# Autodesk Inventor assembly: mearm 期末組合
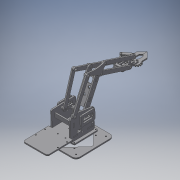
[picture p0: Inventor's stored thumbnail of the model, 180x180]
Saved by Autodesk Inventor 2019 (Build 230136000, 136)
## iProperties
Created: 2022-01-10
Part Number: mearm 期末組合
Material: 一般
Document SubType Name: Assembly
Designer: 10617
Author: 10617
## Documents named in this file (31)
- E:\cad2021\data\tmp\cad2021_hw\downloads\meARM\meARM_Inventor\HW1_mearm零組件\HW1_mearm組合.iam
- E:\cad2021\data\tmp\cad2021_hw\downloads\meARM\meARM_Inventor\HW1_mearm零組件\1.ipt
- E:\cad2021\data\tmp\cad2021_hw\downloads\meARM\meARM_Inventor\HW1_mearm零組件\2.ipt
- E:\cad2021\data\tmp\cad2021_hw\downloads\meARM\meARM_Inventor\HW1_mearm零組件\3.ipt
- E:\cad2021\data\tmp\cad2021_hw\downloads\meARM\meARM_Inventor\HW1_mearm零組件\4.ipt
- E:\cad2021\data\tmp\cad2021_hw\downloads\meARM\meARM_Inventor\HW1_mearm零組件\5.ipt
- E:\cad2021\data\tmp\cad2021_hw\downloads\meARM\meARM_Inventor\HW1_mearm零組件\6.ipt
- E:\cad2021\data\tmp\cad2021_hw\downloads\meARM\meARM_Inventor\HW1_mearm零組件\7.ipt
- E:\cad2021\data\tmp\cad2021_hw\downloads\meARM\meARM_Inventor\HW1_mearm零組件\8.ipt
- E:\cad2021\data\tmp\cad2021_hw\downloads\meARM\meARM_Inventor\HW1_mearm零組件\9.ipt
- E:\cad2021\data\tmp\cad2021_hw\downloads\meARM\meARM_Inventor\HW1_mearm零組件\10.ipt
- E:\cad2021\data\tmp\cad2021_hw\downloads\meARM\meARM_Inventor\HW1_mearm零組件\11.ipt
- E:\cad2021\data\tmp\cad2021_hw\downloads\meARM\meARM_Inventor\HW1_mearm零組件\12.ipt
- E:\cad2021\data\tmp\cad2021_hw\downloads\meARM\meARM_Inventor\HW1_mearm零組件\13.ipt
- E:\cad2021\data\tmp\cad2021_hw\downloads\meARM\meARM_Inventor\HW1_mearm零組件\14.ipt
- E:\cad2021\data\tmp\cad2021_hw\downloads\meARM\meARM_Inventor\HW1_mearm零組件\15.ipt
- E:\cad2021\data\tmp\cad2021_hw\downloads\meARM\meARM_Inventor\HW1_mearm零組件\16.ipt
- E:\cad2021\data\tmp\cad2021_hw\downloads\meARM\meARM_Inventor\HW1_mearm零組件\17.ipt
- E:\cad2021\data\tmp\cad2021_hw\downloads\meARM\meARM_Inventor\HW1_mearm零組件\18.ipt
- E:\cad2021\data\tmp\cad2021_hw\downloads\meARM\meARM_Inventor\HW1_mearm零組件\19.ipt
- E:\cad2021\data\tmp\cad2021_hw\downloads\meARM\meARM_Inventor\HW1_mearm零組件\20.ipt
- E:\cad2021\data\tmp\cad2021_hw\downloads\meARM\meARM_Inventor\HW1_mearm零組件\21.ipt
- E:\cad2021\data\tmp\cad2021_hw\downloads\meARM\meARM_Inventor\HW1_mearm零組件\22.ipt
- E:\cad2021\data\tmp\cad2021_hw\downloads\meARM\meARM_Inventor\HW1_mearm零組件\24.ipt
- E:\cad2021\data\tmp\cad2021_hw\downloads\meARM\meARM_Inventor\HW1_mearm零組件\25.ipt
- E:\cad2021\data\tmp\cad2021_hw\downloads\meARM\meARM_Inventor\HW1_mearm零組件\26.ipt
- E:\cad2021\data\tmp\cad2021_hw\downloads\meARM\meARM_Inventor\HW1_mearm零組件\27.ipt
- E:\cad2021\data\tmp\cad2021_hw\downloads\meARM\meARM_Inventor\HW1_mearm零組件\齒輪.ipt
- E:\cad2021\data\tmp\cad2021_hw\downloads\meARM\meARM_Inventor\HW1_mearm零組件\齒輪2.ipt
- E:\cad2021\data\tmp\cad2021_hw\downloads\meARM\meARM_Inventor\HW1_mearm零組件\23.ipt
- E:\cad2021\data\tmp\cad2021_hw\downloads\meARM\meARM_Inventor\HW1_mearm零組件\軸.ipt
## Components (48 placed, 30 different names)
1. 1:1 — 貼合:105, 貼合:108, 貼合:110, 貼合:117, 齊平:26, 貼合:166, 齊平:33
2. 2:1 — 貼合:106, 貼合:107, 貼合:109, 貼合:111, 貼合:112, 貼合:113, 齊平:22
3. 3:1 — 貼合:101, 貼合:102, 貼合:103, 貼合:104
4. 4:1 — 貼合:119, 貼合:120, 貼合:141
5. 5:1 — 貼合:99, 貼合:100, 貼合:114, 貼合:115, 貼合:163, 齊平:30, 齊平:31
6. 6:1 — 齊平:1, 貼合:1, 貼合:2, 貼合:3, 角度:2, 齊平:3, 貼合:77
7. 7:1 — 角度:2, 齊平:3, 齊平:4, 齊平:5
8. 8:1 — 貼合:86, 貼合:87, 貼合:88
9. 9:1 — 貼合:92, 貼合:93, 貼合:94, 貼合:95, 齊平:14, 貼合:96, 齊平:15
10. 10:1 — 貼合:84, 貼合:85, 齊平:13
11. 11:1 — 貼合:77, 齊平:12, 貼合:78, 貼合:79, 貼合:80, 貼合:81, 貼合:82, 貼合:83, 貼合:165, 齊平:32
12. 12:1 — 貼合:105, 貼合:106, 貼合:107, 貼合:108, 貼合:109, 貼合:110
13. 13:1 — 貼合:103, 貼合:104, 貼合:116, 貼合:118, 貼合:119, 貼合:120, 貼合:156, 齊平:23, 貼合:158, 齊平:25, 貼合:160, 齊平:27
14. 14:1 — 貼合:81, 貼合:82, 貼合:83, 貼合:85, 齊平:13, 貼合:86, 貼合:87, 貼合:88, 貼合:92, 貼合:93, 貼合:94
15. 15:1 — 貼合:116, 貼合:117, 貼合:118, 貼合:140, 貼合:157, 齊平:24
16. 16:1 — 貼合:78, 貼合:79, 貼合:80, 貼合:84, 貼合:89, 貼合:90, 貼合:91, 貼合:101, 貼合:102, 貼合:161, 齊平:28
17. 17:1 — 貼合:89, 貼合:90, 貼合:91
18. 18:1 — 貼合:123, 貼合:125, 貼合:127, 貼合:129, 貼合:142, 貼合:143
19. 19:1 — 貼合:136, 貼合:137, 貼合:139, 貼合:143, 貼合:148, 齊平:17
20. 20:1 — 貼合:97, 貼合:98, 貼合:99, 貼合:100, 貼合:162, 齊平:29, 貼合:164
21. 21:1 — 貼合:95, 齊平:14, 貼合:96, 貼合:97, 貼合:98, 貼合:111, 貼合:112
22. 22:1 — 齊平:1, 貼合:1, 貼合:2, 貼合:3, 齊平:4, 齊平:5, 齊平:12, 齊平:15
23. 24:1 — 貼合:127, 貼合:128, 貼合:129, 貼合:141, 貼合:142, 貼合:154, 齊平:21
24. 25:1 — 貼合:134, 貼合:135, 貼合:136, 貼合:137, 貼合:149, 貼合:150, 貼合:151, 齊平:18
25. 26:1 — 貼合:122, 貼合:123, 貼合:124, 貼合:125, 貼合:126, 貼合:139, 貼合:145, 貼合:146
26. 27:1 — 貼合:113, 貼合:114, 貼合:115, 貼合:140, 貼合:145, 貼合:146, 貼合:147, 齊平:16, 貼合:155
27. 齒輪:1 — 貼合:132, 貼合:133, 貼合:134, 貼合:135, 相切:1
28. 齒輪2:1 — 貼合:130, 貼合:131, 相切:1
29. 23:1 — 貼合:122, 貼合:124, 貼合:126, 貼合:128, 貼合:130, 貼合:131, 貼合:132, 貼合:133, 貼合:152, 齊平:19, 貼合:153, 齊平:20
30. 軸:1 — 貼合:148, 齊平:17
31. 軸:2 — 貼合:149, 貼合:150
32. 軸:3 — 貼合:151, 齊平:18
33. 軸:4 — 貼合:154, 齊平:21
34. 軸:5 — 貼合:157, 齊平:24
35. 軸:6 — 貼合:158, 齊平:25, 貼合:159
36. 軸:7 — 貼合:160, 齊平:27
37. 軸:8 — 貼合:164, 齊平:31
38. 軸:9 — 貼合:153, 齊平:20
39. 軸:10 — 貼合:161, 齊平:28
40. 軸:11 — 貼合:152, 齊平:19
41. 軸:12 — 貼合:163, 齊平:30
42. 軸:13 — 貼合:165, 齊平:32
43. 軸:14 — 貼合:166, 齊平:33
44. 軸:15 — 貼合:162, 齊平:29
45. 軸:16 — 貼合:159, 齊平:26
46. 軸:17 — 貼合:156, 齊平:23
47. 軸:18 — 貼合:155, 齊平:22
48. 軸:19 — 貼合:147, 齊平:16
## Relationships (118: Mate 90, Flush 26, Angle 1, Tangent 1)
- 齊平:1 [Flush] (13 mm): 6:1 ↔ 22:1
- 貼合:1 [Mate]: 6:1 ↔ 22:1
- 貼合:2 [Mate]: 6:1 ↔ 22:1
- 貼合:3 [Mate]: 6:1 ↔ 22:1
- 角度:2 [Angle] (0 deg): 6:1 ↔ 7:1
- 齊平:3 [Flush] (-7.63 mm): 6:1 ↔ 7:1
- 齊平:4 [Flush]: 7:1 ↔ 22:1
- 齊平:5 [Flush]: 7:1 ↔ 22:1
- 貼合:77 [Mate] (-27.48 mm): 6:1 ↔ 11:1
- 齊平:12 [Flush]: 11:1 ↔ 22:1
- 貼合:78 [Mate]: 11:1 ↔ 16:1
- 貼合:79 [Mate]: 11:1 ↔ 16:1
- 貼合:80 [Mate]: 11:1 ↔ 16:1
- 貼合:81 [Mate]: 11:1 ↔ 14:1
- 貼合:82 [Mate]: 11:1 ↔ 14:1
- 貼合:83 [Mate]: 11:1 ↔ 14:1
- 貼合:84 [Mate]: 10:1 ↔ 16:1
- 貼合:85 [Mate]: 10:1 ↔ 14:1
- 齊平:13 [Flush]: 10:1 ↔ 14:1
- 貼合:86 [Mate]: 8:1 ↔ 14:1
- 貼合:87 [Mate]: 8:1 ↔ 14:1
- 貼合:88 [Mate] (2.37 mm): 8:1 ↔ 14:1
- 貼合:89 [Mate]: 16:1 ↔ 17:1
- 貼合:90 [Mate]: 16:1 ↔ 17:1
- 貼合:91 [Mate] (2.37 mm): 16:1 ↔ 17:1
- 貼合:92 [Mate]: 9:1 ↔ 14:1
- 貼合:93 [Mate]: 9:1 ↔ 14:1
- 貼合:94 [Mate]: 9:1 ↔ 14:1
- 貼合:95 [Mate]: 9:1 ↔ 21:1
- 齊平:14 [Flush]: 9:1 ↔ 21:1
- 貼合:96 [Mate]: 9:1 ↔ 21:1
- 貼合:97 [Mate]: 20:1 ↔ 21:1
- 貼合:98 [Mate] (5 mm): 20:1 ↔ 21:1
- 貼合:99 [Mate]: 5:1 ↔ 20:1
- 貼合:100 [Mate] (1.5 mm): 5:1 ↔ 20:1
- 貼合:101 [Mate]: 3:1 ↔ 16:1
- 貼合:102 [Mate]: 3:1 ↔ 16:1
- 貼合:103 [Mate]: 3:1 ↔ 13:1
- 貼合:104 [Mate]: 3:1 ↔ 13:1
- 貼合:105 [Mate]: 1:1 ↔ 12:1
- 貼合:106 [Mate]: 2:1 ↔ 12:1
- 貼合:107 [Mate]: 2:1 ↔ 12:1
- 貼合:108 [Mate]: 1:1 ↔ 12:1
- 貼合:109 [Mate]: 2:1 ↔ 12:1
- 貼合:110 [Mate]: 1:1 ↔ 12:1
- 貼合:111 [Mate]: 2:1 ↔ 21:1
- 貼合:112 [Mate] (0.5 mm): 2:1 ↔ 21:1
- 貼合:113 [Mate]: 2:1 ↔ 27:1
- 貼合:114 [Mate]: 5:1 ↔ 27:1
- 貼合:115 [Mate]: 5:1 ↔ 27:1
- 貼合:116 [Mate]: 13:1 ↔ 15:1
- 貼合:117 [Mate]: 1:1 ↔ 15:1
- 貼合:118 [Mate]: 13:1 ↔ 15:1
- 貼合:119 [Mate]: 4:1 ↔ 13:1
- 貼合:120 [Mate]: 4:1 ↔ 13:1
- 貼合:122 [Mate]: 26:1 ↔ 23:1
- 貼合:123 [Mate]: 18:1 ↔ 26:1
- 貼合:124 [Mate]: 26:1 ↔ 23:1
- 貼合:125 [Mate]: 18:1 ↔ 26:1
- 貼合:126 [Mate]: 26:1 ↔ 23:1
- 貼合:127 [Mate]: 18:1 ↔ 24:1
- 貼合:128 [Mate]: 24:1 ↔ 23:1
- 貼合:129 [Mate]: 18:1 ↔ 24:1
- 齊平:15 [Flush] (6.88 mm): 9:1 ↔ 22:1
- 貼合:130 [Mate]: 齒輪2:1 ↔ 23:1
- 貼合:131 [Mate]: 齒輪2:1 ↔ 23:1
- 貼合:132 [Mate]: 齒輪:1 ↔ 23:1
- 貼合:133 [Mate]: 齒輪:1 ↔ 23:1
- 貼合:134 [Mate]: 25:1 ↔ 齒輪:1
- 貼合:135 [Mate]: 25:1 ↔ 齒輪:1
- 貼合:136 [Mate]: 19:1 ↔ 25:1
- 貼合:137 [Mate] (4.48 mm): 19:1 ↔ 25:1
- 貼合:139 [Mate] (-12 mm): 19:1 ↔ 26:1
- 貼合:140 [Mate]: 15:1 ↔ 27:1
- 貼合:141 [Mate]: 4:1 ↔ 24:1
- 貼合:142 [Mate]: 18:1 ↔ 24:1
- 貼合:143 [Mate] (-11 mm): 18:1 ↔ 19:1
- 貼合:145 [Mate]: 26:1 ↔ 27:1
- 貼合:146 [Mate] (1 mm): 26:1 ↔ 27:1
- 貼合:147 [Mate]: 27:1 ↔ 軸:19
- 齊平:16 [Flush] (-4 mm): 27:1 ↔ 軸:19
- 相切:1 [Tangent]: 齒輪:1 ↔ 齒輪2:1
- 貼合:148 [Mate]: 19:1 ↔ 軸:1
- 齊平:17 [Flush] (-2 mm): 19:1 ↔ 軸:1
- 貼合:149 [Mate]: 25:1 ↔ 軸:2
- 貼合:150 [Mate] (1 mm): 25:1 ↔ 軸:2
- 貼合:151 [Mate]: 25:1 ↔ 軸:3
- 齊平:18 [Flush] (-2 mm): 25:1 ↔ 軸:3
- 貼合:152 [Mate]: 23:1 ↔ 軸:11
- 齊平:19 [Flush] (-2 mm): 23:1 ↔ 軸:11
- 貼合:153 [Mate]: 23:1 ↔ 軸:9
- 齊平:20 [Flush] (-2 mm): 23:1 ↔ 軸:9
- 貼合:154 [Mate]: 24:1 ↔ 軸:4
- 齊平:21 [Flush] (-3 mm): 24:1 ↔ 軸:4
- 貼合:155 [Mate]: 27:1 ↔ 軸:18
- 齊平:22 [Flush] (-1 mm): 2:1 ↔ 軸:18
- 貼合:156 [Mate]: 13:1 ↔ 軸:17
- 齊平:23 [Flush] (2 mm): 13:1 ↔ 軸:17
- 貼合:157 [Mate]: 15:1 ↔ 軸:5
- 齊平:24 [Flush] (-2 mm): 15:1 ↔ 軸:5
- 貼合:158 [Mate]: 13:1 ↔ 軸:6
- 齊平:25 [Flush] (-2 mm): 13:1 ↔ 軸:6
- 貼合:159 [Mate]: 軸:6 ↔ 軸:16
- 齊平:26 [Flush] (-2 mm): 1:1 ↔ 軸:16
- 貼合:160 [Mate]: 13:1 ↔ 軸:7
- 齊平:27 [Flush] (-3 mm): 13:1 ↔ 軸:7
- 貼合:161 [Mate]: 16:1 ↔ 軸:10
- 齊平:28 [Flush] (3 mm): 16:1 ↔ 軸:10
- 貼合:162 [Mate]: 20:1 ↔ 軸:15
- 齊平:29 [Flush] (-1 mm): 20:1 ↔ 軸:15
- 貼合:163 [Mate]: 5:1 ↔ 軸:12
- 齊平:30 [Flush] (-2 mm): 5:1 ↔ 軸:12
- 貼合:164 [Mate]: 20:1 ↔ 軸:8
- 齊平:31 [Flush] (-1 mm): 5:1 ↔ 軸:8
- 貼合:165 [Mate]: 11:1 ↔ 軸:13
- 齊平:32 [Flush] (-4 mm): 11:1 ↔ 軸:13
- 貼合:166 [Mate]: 1:1 ↔ 軸:14
- 齊平:33 [Flush] (-3 mm): 1:1 ↔ 軸:14
